# Autodesk Inventor assembly: makerscannerAssembly
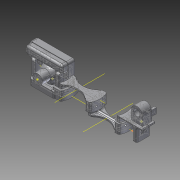
[picture p0: Inventor's stored thumbnail of the model, 180x180]
Saved by Autodesk Inventor 2011 (Build 150239000, 239)
## iProperties
Created: 2010-06-28
Part Number: makerscannerAssembly
Document SubType Name: Assembly
Designer: abarry
Author: abarry
## Documents named in this file (7)
- C:\Users\Sing-E\Documents\abarry\makerscannerAssembly.iam
- C:\Users\Sing-E\Documents\abarry\ps3_eye_assembly2.iam
- C:\Users\Sing-E\Documents\abarry\LaserCameraConnector.ipt
- C:\Users\Sing-E\Documents\abarry\LaserMountBase.ipt
- C:\Users\Sing-E\Documents\abarry\LaserMountPole2.ipt
- C:\Users\Sing-E\Documents\abarry\LaserMountTop.ipt
- C:\Users\Sing-E\Documents\abarry\LaserMountBase2.ipt
## Components (7 placed, 6 different names)
1. ps3_eye_assembly2:1 [sub-assembly] — Flush:3, Flush:4, Flush:5, Mate:9, Mate:10
2. LaserCameraConnector:1 — Flush:3, Flush:4, Mate:7, Mate:8
3. LaserCameraConnector:2 — Flush:6, Mate:7, Mate:8, Flush:7, Mate:15, Mate:16
4. LaserMountBase:1 — Flush:7, Mate:12, Mate:13, Mate:17
5. LaserMountPole2:1 — Mate:12, Mate:13, Mate:14
6. LaserMountTop:1 — Mate:14
7. LaserMountBase2:1 — Mate:15, Mate:16, Mate:17
## Relationships (16: Mate 11, Flush 5)
- Flush:3: ps3_eye_assembly2:1 ↔ LaserCameraConnector:1
- Flush:4 (0.3 mm): ps3_eye_assembly2:1 ↔ LaserCameraConnector:1
- Flush:5: ps3_eye_assembly2:1
- Flush:6: LaserCameraConnector:2
- Mate:7: LaserCameraConnector:1 ↔ LaserCameraConnector:2
- Mate:8: LaserCameraConnector:1 ↔ LaserCameraConnector:2
- Flush:7: LaserCameraConnector:2 ↔ LaserMountBase:1
- Mate:9: ps3_eye_assembly2:1
- Mate:10: ps3_eye_assembly2:1
- Mate:11
- Mate:12: LaserMountBase:1 ↔ LaserMountPole2:1
- Mate:13: LaserMountBase:1 ↔ LaserMountPole2:1
- Mate:14: LaserMountPole2:1 ↔ LaserMountTop:1
- Mate:15: LaserCameraConnector:2 ↔ LaserMountBase2:1
- Mate:16: LaserCameraConnector:2 ↔ LaserMountBase2:1
- Mate:17: LaserMountBase:1 ↔ LaserMountBase2:1
